# Autodesk Inventor assembly: Assembly2
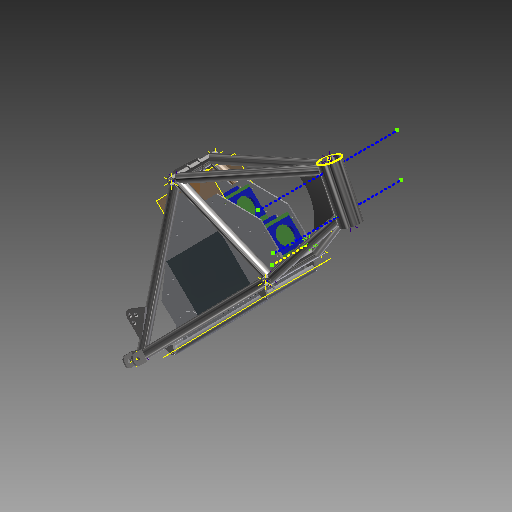
[picture p0: Inventor's stored thumbnail of the model, 512x512]
Saved by Autodesk Inventor 2019.3 (Build 233278000, 278)
## iProperties
Created: 2018-09-28
Part Number: Assembly2
Document SubType Name: Assembly
Designer: eroldan
Author: eroldan
## Documents named in this file (7)
- C:\Users\eroldan\Desktop\3dprojects\OpenEmoto\MainFrame\Battery\Assembly.iam
- C:\Users\eroldan\Desktop\3dprojects\OpenEmoto\MainFrame\MainFrame.ipt
- C:\Users\eroldan\Desktop\3dprojects\OpenEmoto\MainFrame\Battery\LowerCage.ipt
- C:\Users\eroldan\Desktop\3dprojects\OpenEmoto\MainFrame\Battery\BatteryArrangement.iam
- C:\Users\eroldan\Desktop\3dprojects\OpenEmoto\MainFrame\Battery\PlateRight.ipt
- C:\Users\eroldan\Desktop\3dprojects\OpenEmoto\MainFrame\Battery\BMS_JBD-16-20s.ipt
- C:\Users\eroldan\Desktop\3dprojects\OpenEmoto\MainFrame\Battery\LowerPlate.ipt
## Components (7 placed, 6 different names)
1. MainFrame:1 — Flush:1, Flush:2, Mate:1
2. LowerCage:1 — Flush:1, Flush:2, Flush:7, Flush:8, Flush:9, Flush:10
3. BatteryArrangement:1 [sub-assembly] — Mate:1, Flush:4, Mate:4
4. PlateRight:1 — Flush:4, Mate:2, Mate:3, Flush:7, Flush:8, Mate:5
5. PlateRight:2 — Mate:2, Mate:3, Mate:4
6. BMS_JBD-16-20s:1 — Mate:5
7. LowerPlate:1 — Flush:9, Flush:10
## Relationships (12: Flush 7, Mate 5)
- Flush:1: MainFrame:1 ↔ LowerCage:1
- Flush:2: MainFrame:1 ↔ LowerCage:1
- Mate:1: MainFrame:1 ↔ BatteryArrangement:1
- Flush:4: BatteryArrangement:1 ↔ PlateRight:1
- Mate:2: PlateRight:1 ↔ PlateRight:2
- Mate:3: PlateRight:1 ↔ PlateRight:2
- Mate:4: BatteryArrangement:1 ↔ PlateRight:2
- Flush:7: LowerCage:1 ↔ PlateRight:1
- Flush:8: LowerCage:1 ↔ PlateRight:1
- Mate:5: PlateRight:1 ↔ BMS_JBD-16-20s:1
- Flush:9: LowerCage:1 ↔ LowerPlate:1
- Flush:10: LowerCage:1 ↔ LowerPlate:1
